# Autodesk Inventor assembly: Terminal Connector
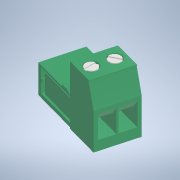
[picture p0: Inventor's stored thumbnail of the model, 180x180]
Saved by Autodesk Inventor 2020 (Build 240168000, 168)
## iProperties
Created: 2019-08-19
Part Number: Terminal Connector
Document SubType Name: Assembly
Designer: SENSE IT OUT
Author: SENSE IT OUT
## Documents named in this file (4)
- E:\Sicca CAD\Control Module_version1.0\Terminal Connector.iam
- E:\Sicca CAD\Control Module_version1.0\Plugin_block.ipt
- E:\Sicca CAD\Control Module_version1.0\plugin_maleblock.ipt
- E:\Sicca CAD\Control Module_version1.0\Screw_Terminal.ipt
## Components (4 placed, 3 different names)
1. Plugin_block:1 — Mate:1, Mate:2, Flush:1, Mate:3, Mate:4, Mate:5, Mate:6
2. plugin_maleblock:1 — Mate:1, Mate:2, Flush:1
3. Screw_Terminal:1 — Mate:3, Mate:6
4. Screw_Terminal:2 — Mate:4, Mate:5
## Relationships (7: Mate 6, Flush 1)
- Mate:1: Plugin_block:1 ↔ plugin_maleblock:1
- Mate:2: Plugin_block:1 ↔ plugin_maleblock:1
- Flush:1: Plugin_block:1 ↔ plugin_maleblock:1
- Mate:3: Plugin_block:1 ↔ Screw_Terminal:1
- Mate:4: Plugin_block:1 ↔ Screw_Terminal:2
- Mate:5: Plugin_block:1 ↔ Screw_Terminal:2
- Mate:6: Plugin_block:1 ↔ Screw_Terminal:1
